# Autodesk Inventor assembly: TPU Based Assembly
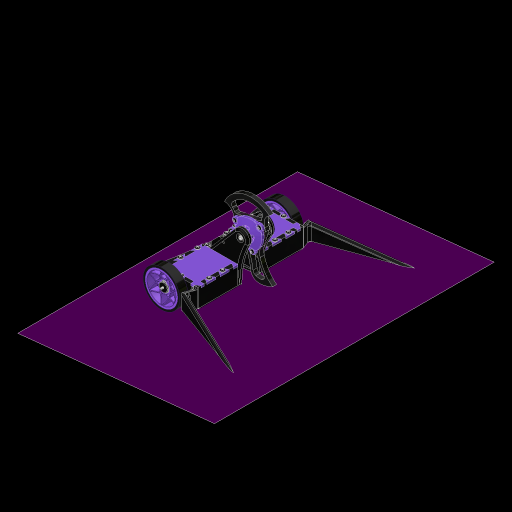
[picture p0: Inventor's stored thumbnail of the model, 512x512]
Saved by Autodesk Inventor 2024.2 (Build 282272000, 272)
## iProperties
Created: 2022-02-23
Part Number: TPU Based Assembly
Document SubType Name: Assembly
Designer: tandu
Mass: 481.188 g
Surface Area: 1600.39 cm^2
Volume: 265.11 cm^3
Density: 1.81505 g/cm^3
Author: tandu
## Documents named in this file (25)
- C:\Users\tandu\Documents\GitHub\GrabCAD\Insomnia 2020\Versions\12 Fixing drive\TPU Based Assembly 12.iam
- C:\Users\tandu\Documents\GitHub\GrabCAD\Insomnia 2020\Versions\12 Fixing drive\BatteryMockup.ipt
- C:\Users\tandu\Documents\GitHub\GrabCAD\Insomnia 2020\Versions\12 Fixing drive\CorrectSizeWheelsIThink.ipt
- C:\Users\tandu\Documents\GitHub\GrabCAD\Insomnia 2020\Versions\12 Fixing drive\EMax RS2205 v1.ipt
- C:\Users\tandu\Documents\GitHub\GrabCAD\Insomnia 2020\Versions\12 Fixing drive\FingerTech_Silver_Spark_223350.ipt
- C:\Users\tandu\Documents\GitHub\GrabCAD\Insomnia 2020\Versions\12 Fixing drive\TPU 22 Chassis.ipt
- C:\Users\tandu\Documents\GitHub\GrabCAD\Insomnia 2020\Versions\12 Fixing drive\UHMWMotorUpright.ipt
- C:\Users\tandu\Documents\GitHub\GrabCAD\Insomnia 2020\Versions\12 Fixing drive\UHMWBearingUpright.ipt
- C:\Users\tandu\Documents\GitHub\GrabCAD\Insomnia 2020\Versions\12 Fixing drive\OldBlade\Aluminimumanfmonfo Jank Weapon Fix.iam
- C:\Users\tandu\Documents\GitHub\GrabCAD\Insomnia 2020\Versions\12 Fixing drive\57155K571_Flanged Ball Bearing.ipt
- C:\Users\tandu\Documents\GitHub\GrabCAD\Insomnia 2020\Versions\12 Fixing drive\2207 5 fixed motor.ipt
- C:\Users\tandu\Documents\GitHub\GrabCAD\Insomnia 2020\Versions\12 Fixing drive\WeaponSpacer.ipt
- C:\Users\tandu\Documents\GitHub\GrabCAD\Insomnia 2020\Versions\12 Fixing drive\Derived Lid v8.ipt
- C:\Users\tandu\Documents\GitHub\GrabCAD\Insomnia 2020\Versions\12 Fixing drive\90417A126_Phillips Rounded Head Thread-Forming Screws.ipt
- E:\Users\tandu\Documents\GrabCAD\Insomnia 2020\Versions\9 Comically Large Weapon 9 28 22\FT Clamping Weapon\Viper-V-Spinner-Add-On.iam
- E:\Users\tandu\Documents\GrabCAD\Insomnia 2020\Versions\9 Comically Large Weapon 9 28 22\TPUWeapon\TPUWeaponAssembly.iam
- C:\Users\tandu\Documents\GitHub\GrabCAD\Insomnia 2020\Versions\12 Fixing drive\AR500 Weapon\AR500 Blade.ipt
- C:\Users\tandu\Documents\GitHub\GrabCAD\Insomnia 2020\Versions\12 Fixing drive\AR500 Weapon\PocketedSymmetrical\Pocketed Symetrical AR500 Blade.ipt
- C:\Users\tandu\Documents\GitHub\GrabCAD\Insomnia 2020\Versions\12 Fixing drive\NewWheels\banebots 3mm hub.iam
- C:\Users\tandu\Documents\GitHub\GrabCAD\Insomnia 2020\Versions\12 Fixing drive\NewWheels\NewWheelCore.ipt
- C:\Users\tandu\Documents\GitHub\GrabCAD\Insomnia 2020\Versions\12 Fixing drive\AR500 Weapon\TPUWeaponHubForAR500Blades.ipt
- C:\Users\tandu\Documents\GitHub\GrabCAD\Insomnia 2020\Versions\12 Fixing drive\AR500 Weapon\Fixed TPU Weapon Hub For AR500 Blades.ipt
- C:\Users\tandu\Documents\GitHub\GrabCAD\Insomnia 2020\Versions\12 Fixing drive\OldBlade\91255A128_Button Head Hex Drive Screw.ipt
- C:\Users\tandu\Documents\GitHub\GrabCAD\Insomnia 2020\Versions\12 Fixing drive\OldBlade\91831A006_18-8 Stainless Steel Nylon-Insert Locknut (1).ipt
- C:\Users\tandu\Documents\GitHub\GrabCAD\Insomnia 2020\Versions\12 Fixing drive\NewWheels\Wide Wheel\WideWheelCore.ipt
## Components (46 placed, 24 different names)
1. BatteryMockup:1 — Mate:1, Mate:6, Mate:7
2. CorrectSizeWheelsIThink:1 — Insert:2
3. FingerTech_Silver_Spark_223350:1 — Insert:9, Mate:4
4. TPU 22 Chassis:1 — Mate:1, Insert:1, Insert:2, Insert:9, Mate:4, Insert:10, Mate:5, Insert:11, Insert:12, Insert:13, Insert:14, Mate:6, Mate:7, Insert:26, Insert:27, Insert:32, Insert:33, Insert:34, Insert:36
5. FingerTech_Silver_Spark_223350:2 — Insert:10, Mate:5
6. CorrectSizeWheelsIThink:2 — Insert:1, Tangent:1
7. UHMWMotorUpright:1 — Insert:11, Insert:12, Insert:15, Insert:16, Insert:23, Insert:24, Symmetry:1, Insert:28, Insert:55
8. UHMWBearingUpright:1 — Insert:13, Insert:14, Insert:22, Symmetry:1, Insert:56
9. EMax RS2205 v1:1 — Insert:15, Insert:16
10. Aluminimumanfmonfo Jank Weapon Fix:1 [sub-assembly] — Insert:25
11. 57155K571_Flanged Ball Bearing:1 — Insert:22
12. 2207 5 fixed motor:1 — Insert:23, Insert:24, Insert:25, Mate:11, Insert:29, Insert:35
13. WeaponSpacer:1
14. Derived Lid v8:1 — Insert:26, Insert:27, Insert:45, Insert:46, Insert:47, Insert:48, Insert:49
15. 90417A126_Phillips Rounded Head Thread-Forming Screws:1 — Insert:28
16. Viper-V-Spinner-Add-On:1 [sub-assembly] — Mate:11, Flush:1
17. TPUWeaponAssembly:1 [sub-assembly] — Insert:29
18. Derived Lid v8:2 — Insert:32, Insert:33, Insert:50, Insert:51, Insert:52, Insert:53, Insert:54
19. AR500 Blade:1 — Mate:21, Mate:22, Mate:23, Insert:37, Insert:38
20. Pocketed Symetrical AR500 Blade:1 — Mate:18, Mate:19, Mate:20, Insert:42, Insert:43, Insert:44
21. banebots 3mm hub:1 [sub-assembly] — Insert:34, Mate:12, Mate:13, Mate:14, Mate:27, Mate:28, Mate:29
22. NewWheelCore:1 — Mate:12, Mate:13, Mate:14, Tangent:2
23. banebots 3mm hub:2 [sub-assembly] — Insert:36, Mate:30, Mate:31, Mate:32
24. NewWheelCore:2
25. TPUWeaponHubForAR500Blades:1 — Insert:35, Mate:18, Mate:19, Mate:20, Mate:21, Mate:22, Mate:23
26. Fixed TPU Weapon Hub For AR500 Blades:1 — Insert:37, Insert:38, Insert:39, Insert:40, Insert:41
27. 91255A128_Button Head Hex Drive Screw:1 — Insert:39
28. 91831A006_18-8 Stainless Steel Nylon-Insert Locknut (1):1 — Insert:42
29. 91831A006_18-8 Stainless Steel Nylon-Insert Locknut (1):2 — Insert:43
30. 91831A006_18-8 Stainless Steel Nylon-Insert Locknut (1):3 — Insert:44
31. 91255A128_Button Head Hex Drive Screw:2 — Insert:41
32. 91255A128_Button Head Hex Drive Screw:3 — Insert:40
33. WideWheelCore:1 — Mate:27, Mate:28, Mate:29
34. WideWheelCore:2 — Mate:30, Mate:31, Mate:32
35. 90417A126_Phillips Rounded Head Thread-Forming Screws:2 — Insert:45
36. 90417A126_Phillips Rounded Head Thread-Forming Screws:3 — Insert:48
37. 90417A126_Phillips Rounded Head Thread-Forming Screws:4 — Insert:46
38. 90417A126_Phillips Rounded Head Thread-Forming Screws:5 — Insert:47
39. 90417A126_Phillips Rounded Head Thread-Forming Screws:6 — Insert:49
40. 90417A126_Phillips Rounded Head Thread-Forming Screws:7 — Insert:50
41. 90417A126_Phillips Rounded Head Thread-Forming Screws:8 — Insert:51
42. 90417A126_Phillips Rounded Head Thread-Forming Screws:9 — Insert:54
43. 90417A126_Phillips Rounded Head Thread-Forming Screws:10 — Insert:53
44. 90417A126_Phillips Rounded Head Thread-Forming Screws:11 — Insert:52
45. 90417A126_Phillips Rounded Head Thread-Forming Screws:12 — Insert:55
46. 90417A126_Phillips Rounded Head Thread-Forming Screws:13 — Insert:56
## Relationships (73: Insert 43, Mate 26, Tangent 2, Symmetry 1, Flush 1)
- Mate:1: BatteryMockup:1 ↔ TPU 22 Chassis:1
- Insert:1: TPU 22 Chassis:1 ↔ CorrectSizeWheelsIThink:2
- Insert:2: CorrectSizeWheelsIThink:1 ↔ TPU 22 Chassis:1
- Insert:9: FingerTech_Silver_Spark_223350:1 ↔ TPU 22 Chassis:1
- Mate:4: FingerTech_Silver_Spark_223350:1 ↔ TPU 22 Chassis:1
- Insert:10: TPU 22 Chassis:1 ↔ FingerTech_Silver_Spark_223350:2
- Mate:5: TPU 22 Chassis:1 ↔ FingerTech_Silver_Spark_223350:2
- Insert:11: TPU 22 Chassis:1 ↔ UHMWMotorUpright:1
- Insert:12: TPU 22 Chassis:1 ↔ UHMWMotorUpright:1
- Insert:13: TPU 22 Chassis:1 ↔ UHMWBearingUpright:1
- Insert:14: TPU 22 Chassis:1 ↔ UHMWBearingUpright:1
- Insert:15: UHMWMotorUpright:1 ↔ EMax RS2205 v1:1
- Insert:16: UHMWMotorUpright:1 ↔ EMax RS2205 v1:1
- Insert:22: UHMWBearingUpright:1 ↔ 57155K571_Flanged Ball Bearing:1
- Insert:23: UHMWMotorUpright:1 ↔ 2207 5 fixed motor:1
- Insert:24: UHMWMotorUpright:1 ↔ 2207 5 fixed motor:1
- Insert:25: Aluminimumanfmonfo Jank Weapon Fix:1 ↔ 2207 5 fixed motor:1
- Mate:6: BatteryMockup:1 ↔ TPU 22 Chassis:1
- Mate:7: BatteryMockup:1 ↔ TPU 22 Chassis:1
- Symmetry:1: UHMWMotorUpright:1 ↔ UHMWBearingUpright:1
- Mate:10
- Tangent:1: CorrectSizeWheelsIThink:2
- Insert:26: TPU 22 Chassis:1 ↔ Derived Lid v8:1
- Insert:27: TPU 22 Chassis:1 ↔ Derived Lid v8:1
- Insert:28: UHMWMotorUpright:1 ↔ 90417A126_Phillips Rounded Head Thread-Forming Screws:1
- Mate:11: 2207 5 fixed motor:1 ↔ Viper-V-Spinner-Add-On:1
- Flush:1: Viper-V-Spinner-Add-On:1
- Insert:29: 2207 5 fixed motor:1 ↔ TPUWeaponAssembly:1
- Insert:32: TPU 22 Chassis:1 ↔ Derived Lid v8:2
- Insert:33: TPU 22 Chassis:1 ↔ Derived Lid v8:2
- Insert:34: TPU 22 Chassis:1 ↔ banebots 3mm hub:1
- Mate:12: banebots 3mm hub:1 ↔ NewWheelCore:1
- Mate:13: banebots 3mm hub:1 ↔ NewWheelCore:1
- Mate:14: banebots 3mm hub:1 ↔ NewWheelCore:1
- [Mate]: banebots 3mm hub:2 ↔ NewWheelCore:2
- [Mate]: banebots 3mm hub:2 ↔ NewWheelCore:2
- [Mate]: banebots 3mm hub:2 ↔ NewWheelCore:2
- Insert:35: 2207 5 fixed motor:1 ↔ TPUWeaponHubForAR500Blades:1
- Mate:18: Pocketed Symetrical AR500 Blade:1 ↔ TPUWeaponHubForAR500Blades:1
- Mate:19: Pocketed Symetrical AR500 Blade:1 ↔ TPUWeaponHubForAR500Blades:1
- Insert:36: TPU 22 Chassis:1 ↔ banebots 3mm hub:2
- Mate:20: Pocketed Symetrical AR500 Blade:1 ↔ TPUWeaponHubForAR500Blades:1
- Mate:21: AR500 Blade:1 ↔ TPUWeaponHubForAR500Blades:1
- Mate:22: AR500 Blade:1 ↔ TPUWeaponHubForAR500Blades:1
- Mate:23: AR500 Blade:1 ↔ TPUWeaponHubForAR500Blades:1
- Insert:37: AR500 Blade:1 ↔ Fixed TPU Weapon Hub For AR500 Blades:1
- Insert:38: AR500 Blade:1 ↔ Fixed TPU Weapon Hub For AR500 Blades:1
- Mate:26
- Tangent:2: NewWheelCore:1
- Insert:39: Fixed TPU Weapon Hub For AR500 Blades:1 ↔ 91255A128_Button Head Hex Drive Screw:1
- Insert:40: Fixed TPU Weapon Hub For AR500 Blades:1 ↔ 91255A128_Button Head Hex Drive Screw:3
- Insert:41: Fixed TPU Weapon Hub For AR500 Blades:1 ↔ 91255A128_Button Head Hex Drive Screw:2
- Insert:42: Pocketed Symetrical AR500 Blade:1 ↔ 91831A006_18-8 Stainless Steel Nylon-Insert Locknut (1):1
- Insert:43: Pocketed Symetrical AR500 Blade:1 ↔ 91831A006_18-8 Stainless Steel Nylon-Insert Locknut (1):2
- Insert:44: Pocketed Symetrical AR500 Blade:1 ↔ 91831A006_18-8 Stainless Steel Nylon-Insert Locknut (1):3
- Mate:27: banebots 3mm hub:1 ↔ WideWheelCore:1
- Mate:28: banebots 3mm hub:1 ↔ WideWheelCore:1
- Mate:29: banebots 3mm hub:1 ↔ WideWheelCore:1
- Mate:30: banebots 3mm hub:2 ↔ WideWheelCore:2
- Mate:31: banebots 3mm hub:2 ↔ WideWheelCore:2
- Mate:32: banebots 3mm hub:2 ↔ WideWheelCore:2
- Insert:45: Derived Lid v8:1 ↔ 90417A126_Phillips Rounded Head Thread-Forming Screws:2
- Insert:46: Derived Lid v8:1 ↔ 90417A126_Phillips Rounded Head Thread-Forming Screws:4
- Insert:47: Derived Lid v8:1 ↔ 90417A126_Phillips Rounded Head Thread-Forming Screws:5
- Insert:48: Derived Lid v8:1 ↔ 90417A126_Phillips Rounded Head Thread-Forming Screws:3
- Insert:49: Derived Lid v8:1 ↔ 90417A126_Phillips Rounded Head Thread-Forming Screws:6
- Insert:50: Derived Lid v8:2 ↔ 90417A126_Phillips Rounded Head Thread-Forming Screws:7
- Insert:51: Derived Lid v8:2 ↔ 90417A126_Phillips Rounded Head Thread-Forming Screws:8
- Insert:52: Derived Lid v8:2 ↔ 90417A126_Phillips Rounded Head Thread-Forming Screws:11
- Insert:53: Derived Lid v8:2 ↔ 90417A126_Phillips Rounded Head Thread-Forming Screws:10
- Insert:54: Derived Lid v8:2 ↔ 90417A126_Phillips Rounded Head Thread-Forming Screws:9
- Insert:55: UHMWMotorUpright:1 ↔ 90417A126_Phillips Rounded Head Thread-Forming Screws:12
- Insert:56: UHMWBearingUpright:1 ↔ 90417A126_Phillips Rounded Head Thread-Forming Screws:13
## Named parameters: d69_d66 = 0 mm, d70_d67 = 0 mm, d71_d68 = 0 mm
